# Autodesk Inventor assembly: NDV-2000 Collector 01
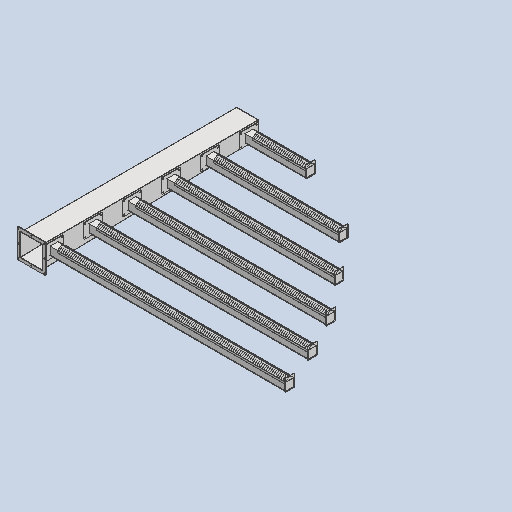
[picture p0: Inventor's stored thumbnail of the model, 512x512]
Saved by Autodesk Inventor 2026.2 (Build 302298000, 298)
## iProperties
Created: 2026-05-12
Part Number: NDV-2000 Collector 01
Document SubType Name: Assembly
Designer: admin
Stock Number: Коллектор
Author: admin
## Documents named in this file (11)
- C:\Users\admin\Documents\Inventor\NDV-DistribSystem\DRS_D1200\NDV-2000 Collector 01.iam
- C:\Users\admin\Documents\Inventor\NDV-DistribSystem\DRS_D1200\NDV-2102 Collector top 01.ipt
- C:\Users\admin\Documents\Inventor\NDV-DistribSystem\DRS_D1200\NDV-2101 Collector bottom 01.ipt
- C:\Users\admin\Documents\Inventor\NDV-DistribSystem\DRS_D1200\NDV-2104 Collector cap 01.ipt
- C:\Users\admin\Documents\Inventor\NDV-DistribSystem\DRS_D1200\NDV-2103 Collector flange 01.ipt
- C:\Users\admin\Documents\Inventor\NDV-DistribSystem\DRS_D1200\NDV-3100 Branch 1 01.iam
- C:\Users\admin\Documents\Inventor\NDV-DistribSystem\DRS_D1200\NDV-3200 Branch 2 01.iam
- C:\Users\admin\Documents\Inventor\NDV-DistribSystem\DRS_D1200\NDV-3300 Branch 3 01.iam
- C:\Users\admin\Documents\Inventor\NDV-DistribSystem\DRS_D1200\NDV-3400 Branch 4 01.iam
- C:\Users\admin\Documents\Inventor\NDV-DistribSystem\DRS_D1200\NDV-3500 Branch 5 01.iam
- C:\Users\admin\Documents\Inventor\NDV-DistribSystem\DRS_D1200\NDV-3600 Branch 6 01.iam
## Components (10 placed, 10 different names)
1. NDV-2102 Collector top 01:1 — Flush:10, Flush:9, Mate:11, Rigid:23, Mate:108
2. NDV-2101 Collector bottom 01:1 — Rigid:23, Mate:107, Flush:43, Mate:109, Mate:110, Mate:111, Mate:112, Mate:113, Mate:114, Mate:115, Mate:116, Mate:117, Mate:118, Mate:119, Mate:120, Mate:121, Mate:122, Mate:123, Mate:124, Mate:125, Mate:126
3. NDV-2104 Collector cap 01:1 — Flush:10, Flush:9, Mate:11
4. NDV-2103 Collector flange 01:1 — Mate:107, Mate:108, Flush:43
5. NDV-3100 Branch 1 01:1 [sub-assembly] — Mate:109, Mate:110, Mate:111
6. NDV-3200 Branch 2 01:1 [sub-assembly] — Mate:112, Mate:113, Mate:114
7. NDV-3300 Branch 3 01:1 [sub-assembly] — Mate:115, Mate:116, Mate:117
8. NDV-3400 Branch 4 01:1 [sub-assembly] — Mate:118, Mate:119, Mate:120
9. NDV-3500 Branch 5 01:1 [sub-assembly] — Mate:121, Mate:122, Mate:123
10. NDV-3600 Branch 6 01:1 [sub-assembly] — Mate:124, Mate:125, Mate:126
## Relationships (25: Mate 21, Flush 3, WeldJoint 1)
- Flush:10 (1 mm): NDV-2102 Collector top 01:1 ↔ NDV-2104 Collector cap 01:1
- Flush:9 (-1 mm): NDV-2102 Collector top 01:1 ↔ NDV-2104 Collector cap 01:1
- Mate:11: NDV-2102 Collector top 01:1 ↔ NDV-2104 Collector cap 01:1
- Rigid:23 [WeldJoint]: NDV-2102 Collector top 01:1 ↔ NDV-2101 Collector bottom 01:1
- Mate:107 (1.1 mm): NDV-2101 Collector bottom 01:1 ↔ NDV-2103 Collector flange 01:1
- Mate:108 (0.1 mm): NDV-2102 Collector top 01:1 ↔ NDV-2103 Collector flange 01:1
- Flush:43: NDV-2101 Collector bottom 01:1 ↔ NDV-2103 Collector flange 01:1
- Mate:109: NDV-2101 Collector bottom 01:1 ↔ NDV-3100 Branch 1 01:1
- Mate:110 (0.25 mm): NDV-2101 Collector bottom 01:1 ↔ NDV-3100 Branch 1 01:1
- Mate:111 (0.25 mm): NDV-2101 Collector bottom 01:1 ↔ NDV-3100 Branch 1 01:1
- Mate:112: NDV-2101 Collector bottom 01:1 ↔ NDV-3200 Branch 2 01:1
- Mate:113 (0.25 mm): NDV-2101 Collector bottom 01:1 ↔ NDV-3200 Branch 2 01:1
- Mate:114 (0.25 mm): NDV-2101 Collector bottom 01:1 ↔ NDV-3200 Branch 2 01:1
- Mate:115: NDV-2101 Collector bottom 01:1 ↔ NDV-3300 Branch 3 01:1
- Mate:116 (0.25 mm): NDV-2101 Collector bottom 01:1 ↔ NDV-3300 Branch 3 01:1
- Mate:117 (0.25 mm): NDV-2101 Collector bottom 01:1 ↔ NDV-3300 Branch 3 01:1
- Mate:118: NDV-2101 Collector bottom 01:1 ↔ NDV-3400 Branch 4 01:1
- Mate:119 (0.25 mm): NDV-2101 Collector bottom 01:1 ↔ NDV-3400 Branch 4 01:1
- Mate:120 (0.25 mm): NDV-2101 Collector bottom 01:1 ↔ NDV-3400 Branch 4 01:1
- Mate:121: NDV-2101 Collector bottom 01:1 ↔ NDV-3500 Branch 5 01:1
- Mate:122 (0.25 mm): NDV-2101 Collector bottom 01:1 ↔ NDV-3500 Branch 5 01:1
- Mate:123 (0.25 mm): NDV-2101 Collector bottom 01:1 ↔ NDV-3500 Branch 5 01:1
- Mate:124: NDV-2101 Collector bottom 01:1 ↔ NDV-3600 Branch 6 01:1
- Mate:125 (0.25 mm): NDV-2101 Collector bottom 01:1 ↔ NDV-3600 Branch 6 01:1
- Mate:126 (0.25 mm): NDV-2101 Collector bottom 01:1 ↔ NDV-3600 Branch 6 01:1
